# Autodesk Inventor assembly: Leg_joint
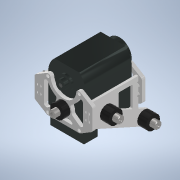
[picture p0: Inventor's stored thumbnail of the model, 180x180]
Saved by Autodesk Inventor 2020.4 (Build 244396000, 396)
## iProperties
Created: 2021-09-06
Part Number: Leg_joint
Document SubType Name: Assembly
Designer: Masato
Mass: 155.537 g
Surface Area: 333.044 cm^2
Volume: 75.5065 cm^3
Density: 2.05992 g/cm^3
Author: Masato
## Documents named in this file (11)
- C:\Users\Masato\Desktop\OpenPlatform_ver3_0\LowerBody\付け根\Leg_joint.iam
- C:\Users\Masato\Desktop\OpenPlatform_ver3_0\LowerBody\付け根\Leg_Joint_side_frame.ipt
- C:\Users\Masato\Desktop\OpenPlatform_ver3_0\LowerBody\付け根\Leg_Joint_backfront_frame.ipt
- C:\Users\Masato\Desktop\OpenPlatform_ver3_0\Ready_Made\B3M11xx.ipt
- C:\Users\Masato\Desktop\OpenPlatform_ver3_0\Ready_Made\SLSBF6-39_5-M3-N3.ipt
- C:\Users\Masato\Desktop\OpenPlatform_ver3_0\Ready_Made\UUW-0312-10BH.ipt
- C:\Users\Masato\Desktop\OpenPlatform_ver3_0\Ready_Made\S3-07-3W.ipt
- C:\Users\Masato\Desktop\OpenPlatform_ver3_0\Ready_Made\CC-0612-25B.ipt
- C:\Users\Masato\Desktop\OpenPlatform_ver3_0\Ready_Made\CC-0612-20B.ipt
- C:\Users\Masato\Desktop\OpenPlatform_ver3_0\Ready_Made\BRU-311S.ipt
- C:\Users\Masato\Desktop\OpenPlatform_ver3_0\Ready_Made\ARU-309S.ipt
## Components (36 placed, 10 different names)
1. Leg_Joint_side_frame:1 — メイト:1, メイト:2, フラッシュ:1, 挿入:11, 挿入:27, 挿入:28, 挿入:45
2. Leg_Joint_side_frame:2 — メイト:3, メイト:4, フラッシュ:2, 挿入:12, 挿入:25, 挿入:26, 挿入:46
3. Leg_Joint_backfront_frame:1 — 挿入:3, 挿入:4, 挿入:5, 挿入:6, メイト:1, メイト:2, フラッシュ:1, メイト:3, メイト:4, フラッシュ:2, 挿入:81
4. Leg_Joint_backfront_frame:2 — 挿入:7, 挿入:8, 挿入:9, 挿入:10, 挿入:55
5. B3M11xx:1 — 挿入:3, 挿入:4, 挿入:5, 挿入:6, 挿入:7, 挿入:8, 挿入:9, 挿入:10, フラッシュ:6, メイト:8, メイト:10
6. SLSBF6-39_5-M3-N3:1 — 挿入:11, 挿入:12
7. UUW-0312-10BH:1 — 挿入:27, 挿入:83, 挿入:100
8. UUW-0312-10BH:2 — 挿入:28, 挿入:82, 挿入:101
9. UUW-0312-10BH:3 — 挿入:25, 挿入:90, 挿入:99
10. UUW-0312-10BH:4 — 挿入:26, 挿入:93, 挿入:98
11. S3-07-3W:1 — 挿入:45
12. S3-07-3W:2 — 挿入:46
13. UUW-0312-10BH:5 — 挿入:55, 挿入:96, 挿入:103
14. UUW-0312-10BH:6 — 挿入:81, 挿入:84, 挿入:102
15. CC-0612-25B:1 — 挿入:82, 挿入:88
16. CC-0612-25B:2 — 挿入:83, 挿入:86
17. CC-0612-25B:3 — 挿入:90, 挿入:91
18. CC-0612-25B:4 — 挿入:93, 挿入:94
19. CC-0612-25B:5 — 挿入:96, 挿入:97
20. CC-0612-25B:6 — 挿入:84, 挿入:85
21. CC-0612-20B:1 — 挿入:88, 挿入:89
22. CC-0612-20B:2 — 挿入:86, 挿入:87
23. CC-0612-20B:3 — 挿入:85
24. CC-0612-20B:4 — 挿入:92
25. CC-0612-20B:5 — 挿入:94, 挿入:95
26. CC-0612-20B:6 — 挿入:97
27. CC-0612-20B:7 — 挿入:89
28. CC-0612-20B:8 — 挿入:87
29. CC-0612-20B:9 — 挿入:91, 挿入:92
30. CC-0612-20B:10 — 挿入:95
31. BRU-311S:1 — 挿入:99
32. BRU-311S:2 — 挿入:98
33. BRU-311S:3 — 挿入:101
34. BRU-311S:4 — 挿入:100
35. ARU-309S:1 — 挿入:102
36. ARU-309S:2 — 挿入:103
## Relationships (49: Insert 40, Mate 6, Flush 3)
- 挿入:3 [Insert]: Leg_Joint_backfront_frame:1 ↔ B3M11xx:1
- 挿入:4 [Insert]: Leg_Joint_backfront_frame:1 ↔ B3M11xx:1
- 挿入:5 [Insert]: Leg_Joint_backfront_frame:1 ↔ B3M11xx:1
- 挿入:6 [Insert]: Leg_Joint_backfront_frame:1 ↔ B3M11xx:1
- 挿入:7 [Insert]: Leg_Joint_backfront_frame:2 ↔ B3M11xx:1
- 挿入:8 [Insert]: Leg_Joint_backfront_frame:2 ↔ B3M11xx:1
- 挿入:9 [Insert]: Leg_Joint_backfront_frame:2 ↔ B3M11xx:1
- 挿入:10 [Insert]: Leg_Joint_backfront_frame:2 ↔ B3M11xx:1
- メイト:1 [Mate] (0.01 mm): Leg_Joint_side_frame:1 ↔ Leg_Joint_backfront_frame:1
- メイト:2 [Mate] (0.01 mm): Leg_Joint_side_frame:1 ↔ Leg_Joint_backfront_frame:1
- フラッシュ:1 [Flush]: Leg_Joint_side_frame:1 ↔ Leg_Joint_backfront_frame:1
- メイト:3 [Mate] (0.01 mm): Leg_Joint_side_frame:2 ↔ Leg_Joint_backfront_frame:1
- メイト:4 [Mate] (0.01 mm): Leg_Joint_side_frame:2 ↔ Leg_Joint_backfront_frame:1
- フラッシュ:2 [Flush]: Leg_Joint_side_frame:2 ↔ Leg_Joint_backfront_frame:1
- 挿入:11 [Insert]: Leg_Joint_side_frame:1 ↔ SLSBF6-39_5-M3-N3:1
- 挿入:12 [Insert]: Leg_Joint_side_frame:2 ↔ SLSBF6-39_5-M3-N3:1
- 挿入:25 [Insert]: Leg_Joint_side_frame:2 ↔ UUW-0312-10BH:3
- 挿入:26 [Insert]: Leg_Joint_side_frame:2 ↔ UUW-0312-10BH:4
- 挿入:27 [Insert]: Leg_Joint_side_frame:1 ↔ UUW-0312-10BH:1
- 挿入:28 [Insert]: Leg_Joint_side_frame:1 ↔ UUW-0312-10BH:2
- フラッシュ:6 [Flush]: B3M11xx:1
- メイト:8 [Mate]: B3M11xx:1
- 挿入:45 [Insert]: Leg_Joint_side_frame:1 ↔ S3-07-3W:1
- 挿入:46 [Insert]: Leg_Joint_side_frame:2 ↔ S3-07-3W:2
- 挿入:55 [Insert]: Leg_Joint_backfront_frame:2 ↔ UUW-0312-10BH:5
- メイト:10 [Mate]: B3M11xx:1
- 挿入:81 [Insert]: Leg_Joint_backfront_frame:1 ↔ UUW-0312-10BH:6
- 挿入:82 [Insert]: UUW-0312-10BH:2 ↔ CC-0612-25B:1
- 挿入:83 [Insert]: UUW-0312-10BH:1 ↔ CC-0612-25B:2
- 挿入:84 [Insert]: UUW-0312-10BH:6 ↔ CC-0612-25B:6
- 挿入:85 [Insert]: CC-0612-25B:6 ↔ CC-0612-20B:3
- 挿入:86 [Insert]: CC-0612-25B:2 ↔ CC-0612-20B:2
- 挿入:87 [Insert]: CC-0612-20B:2 ↔ CC-0612-20B:8
- 挿入:88 [Insert]: CC-0612-25B:1 ↔ CC-0612-20B:1
- 挿入:89 [Insert]: CC-0612-20B:1 ↔ CC-0612-20B:7
- 挿入:90 [Insert]: UUW-0312-10BH:3 ↔ CC-0612-25B:3
- 挿入:91 [Insert]: CC-0612-25B:3 ↔ CC-0612-20B:9
- 挿入:92 [Insert]: CC-0612-20B:4 ↔ CC-0612-20B:9
- 挿入:93 [Insert]: UUW-0312-10BH:4 ↔ CC-0612-25B:4
- 挿入:94 [Insert]: CC-0612-25B:4 ↔ CC-0612-20B:5
- 挿入:95 [Insert]: CC-0612-20B:5 ↔ CC-0612-20B:10
- 挿入:96 [Insert]: UUW-0312-10BH:5 ↔ CC-0612-25B:5
- 挿入:97 [Insert]: CC-0612-25B:5 ↔ CC-0612-20B:6
- 挿入:98 [Insert]: UUW-0312-10BH:4 ↔ BRU-311S:2
- 挿入:99 [Insert]: UUW-0312-10BH:3 ↔ BRU-311S:1
- 挿入:100 [Insert]: UUW-0312-10BH:1 ↔ BRU-311S:4
- 挿入:101 [Insert]: UUW-0312-10BH:2 ↔ BRU-311S:3
- 挿入:102 [Insert]: UUW-0312-10BH:6 ↔ ARU-309S:1
- 挿入:103 [Insert]: UUW-0312-10BH:5 ↔ ARU-309S:2
